# Autodesk Inventor assembly: outer_mirrored
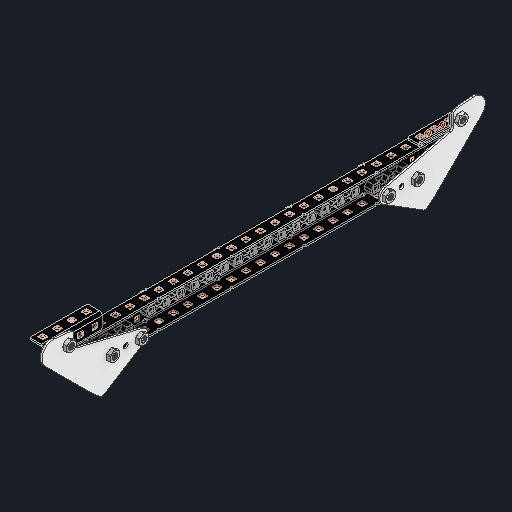
[picture p0: Inventor's stored thumbnail of the model, 512x512]
Saved by Autodesk Inventor 2024 (Build 280153000, 153)
## iProperties
Created: 2024-03-21
Part Number: outer_mirrored
Document SubType Name: Assembly
Designer: Averey Ku
Author: Averey Ku
## Documents named in this file (9)
- D:\vex_robotics\hardware\cad\infection\chassis\mirrored_parts\outer_mirrored.iam
- D:\vex_robotics\hardware\cad\infection\chassis\mirrored_parts\Bearing Flat Low Profile_mirrored.ipt
- D:\vex_robotics\hardware\cad\infection\chassis\mirrored_parts\sled_mirrored.ipt
- D:\vex_robotics\hardware\cad\infection\chassis\mirrored_parts\Nut Nylon Thread Forming_mirrored.ipt
- D:\vex_robotics\hardware\cad\infection\chassis\mirrored_parts\Alu Angle 1x1x4_mirrored.ipt
- D:\vex_robotics\hardware\cad\VEX-CAD-Inventor-1.41\Structure\Standoff\Standoff .875.ipt
- D:\vex_robotics\hardware\cad\VEX-CAD-Inventor-1.41\Structure\Standoff.ipt
- D:\vex_robotics\hardware\cad\infection\chassis\mirrored_parts\Alu C 1x2x1x26_mirrored.ipt
- D:\vex_robotics\hardware\cad\infection\chassis\mirrored_parts\sled_l_channel_mirrored.ipt
## Components (20 placed, 7 different names)
1. Bearing Flat Low Profile_mirrored:1 — Mate:25, Mate:16, Insert:27
2. Bearing Flat Low Profile_mirrored:2 — Mate:18, Insert:29
3. Bearing Flat Low Profile_mirrored:3 — Mate:15, Mate:21, Insert:33
4. Bearing Flat Low Profile_mirrored:4 — Mate:20, Insert:32
5. Bearing Flat Low Profile_mirrored:5 — Mate:19, Insert:31
6. Bearing Flat Low Profile_mirrored:6 — Insert:30
7. Bearing Flat Low Profile_mirrored:7 — Mate:17, Insert:28
8. sled_mirrored:1 — Mate:25, Insert:26, Insert:15, Insert:14, Insert:35
9. sled_mirrored:2 — Mate:15, Insert:24, Insert:17, Insert:18, Insert:25
10. Nut Nylon Thread Forming_mirrored:1 — Insert:26
11. Nut Nylon Thread Forming_mirrored:2 — Insert:15
12. Nut Nylon Thread Forming_mirrored:3 — Insert:14
13. Alu Angle 1x1x4_mirrored:1 — Insert:24, Mate:23, Mate:22
14. Nut Nylon Thread Forming_mirrored:4 — Insert:17
15. Nut Nylon Thread Forming_mirrored:5 — Insert:18
16. Nut Nylon Thread Forming_mirrored:6 — Insert:25
17. Standoff .875:1
18. Standoff .875:2
19. Alu C 1x2x1x26_mirrored:1 — Mate:23, Mate:22, Mate:21, Insert:33, Mate:20, Insert:32, Mate:19, Insert:31, Insert:30, Mate:18, Insert:29, Mate:17, Insert:28, Mate:16, Insert:27, Mate:26, Insert:34
20. sled_l_channel_mirrored:1 — Insert:35, Mate:26, Insert:34
## Relationships (27: Insert 16, Mate 11)
- Mate:25: Bearing Flat Low Profile_mirrored:1 ↔ sled_mirrored:1
- Mate:15: Bearing Flat Low Profile_mirrored:3 ↔ sled_mirrored:2
- Insert:26: sled_mirrored:1 ↔ Nut Nylon Thread Forming_mirrored:1
- Insert:15: sled_mirrored:1 ↔ Nut Nylon Thread Forming_mirrored:2
- Insert:14: sled_mirrored:1 ↔ Nut Nylon Thread Forming_mirrored:3
- Insert:24: sled_mirrored:2 ↔ Alu Angle 1x1x4_mirrored:1
- Insert:17: sled_mirrored:2 ↔ Nut Nylon Thread Forming_mirrored:4
- Insert:18: sled_mirrored:2 ↔ Nut Nylon Thread Forming_mirrored:5
- Insert:25: sled_mirrored:2 ↔ Nut Nylon Thread Forming_mirrored:6
- Mate:23: Alu Angle 1x1x4_mirrored:1 ↔ Alu C 1x2x1x26_mirrored:1
- Mate:22: Alu Angle 1x1x4_mirrored:1 ↔ Alu C 1x2x1x26_mirrored:1
- Mate:21: Bearing Flat Low Profile_mirrored:3 ↔ Alu C 1x2x1x26_mirrored:1
- Insert:33: Bearing Flat Low Profile_mirrored:3 ↔ Alu C 1x2x1x26_mirrored:1
- Mate:20: Bearing Flat Low Profile_mirrored:4 ↔ Alu C 1x2x1x26_mirrored:1
- Insert:32: Bearing Flat Low Profile_mirrored:4 ↔ Alu C 1x2x1x26_mirrored:1
- Mate:19: Bearing Flat Low Profile_mirrored:5 ↔ Alu C 1x2x1x26_mirrored:1
- Insert:31: Bearing Flat Low Profile_mirrored:5 ↔ Alu C 1x2x1x26_mirrored:1
- Insert:30: Bearing Flat Low Profile_mirrored:6 ↔ Alu C 1x2x1x26_mirrored:1
- Mate:18: Bearing Flat Low Profile_mirrored:2 ↔ Alu C 1x2x1x26_mirrored:1
- Insert:29: Bearing Flat Low Profile_mirrored:2 ↔ Alu C 1x2x1x26_mirrored:1
- Mate:17: Bearing Flat Low Profile_mirrored:7 ↔ Alu C 1x2x1x26_mirrored:1
- Insert:28: Bearing Flat Low Profile_mirrored:7 ↔ Alu C 1x2x1x26_mirrored:1
- Mate:16: Bearing Flat Low Profile_mirrored:1 ↔ Alu C 1x2x1x26_mirrored:1
- Insert:27: Bearing Flat Low Profile_mirrored:1 ↔ Alu C 1x2x1x26_mirrored:1
- Insert:35: sled_mirrored:1 ↔ sled_l_channel_mirrored:1
- Mate:26: Alu C 1x2x1x26_mirrored:1 ↔ sled_l_channel_mirrored:1
- Insert:34: Alu C 1x2x1x26_mirrored:1 ↔ sled_l_channel_mirrored:1
